# Autodesk Inventor assembly: Rotating Assembly
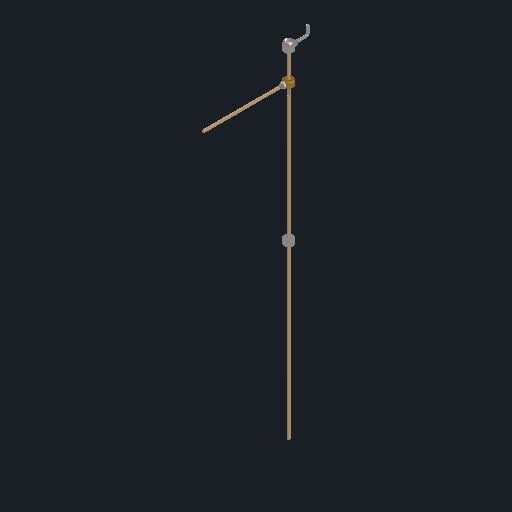
[picture p0: Inventor's stored thumbnail of the model, 512x512]
Saved by Autodesk Inventor 2027.1 (Build 311270010, 270A)
## iProperties
Created: 2025-09-16
Document SubType Name: Assembly
Designer: SD
Mass: 42.3595 g
Surface Area: 61.7875 cm^2
Volume: 4.97569 cm^3
Density: 8.51329 g/cm^3
Project: Automatic Tea Steeping mechanism
Part Number: Rotating Assembly
BOM-Mass: 0.04236
BOM-Area: 0.006
Author: SD
Title: Rotating Assembly
## Documents named in this file (9)
- C:\Users\Gamer\Documents\Projects\Auto Tea Steeper\Public Version\Automatic Tea Steeper\CAD\Workspace\Rotating Assembly.iam
- C:\Users\Gamer\Documents\Projects\Auto Tea Steeper\Public Version\Automatic Tea Steeper\CAD\Workspace\Rotating Rod 370mm.ipt
- C:\Users\Gamer\Documents\Projects\Auto Tea Steeper\Public Version\Automatic Tea Steeper\CAD\Workspace\Top Lock Cap.ipt
- C:\Users\Gamer\Documents\Projects\Auto Tea Steeper\Public Version\Automatic Tea Steeper\CAD\Workspace\Lock Handel.ipt
- C:\Users\Gamer\Documents\Projects\Auto Tea Steeper\Public Version\Automatic Tea Steeper\CAD\Workspace\Hardware\M3 Hex Nut.ipt
- C:\Users\Gamer\Documents\Projects\Auto Tea Steeper\Public Version\Automatic Tea Steeper\CAD\Workspace\Pendulum Arm Cap.ipt
- C:\Users\Gamer\Documents\Projects\Auto Tea Steeper\Public Version\Automatic Tea Steeper\CAD\Workspace\Pendulum Arm.ipt
- C:\Users\Gamer\Documents\Projects\Auto Tea Steeper\Public Version\Automatic Tea Steeper\CAD\Workspace\Lower Lock Cap.ipt
- C:\Users\Gamer\Documents\Projects\Auto Tea Steeper\Public Version\Automatic Tea Steeper\CAD\Workspace\Hardware\Grub Screw 3x3mm.ipt
## Components (9 placed, 8 different names)
1. Rotating Rod 370mm:1 — Flush:1, Mate:1, Mate:2, Mate:5, Mate:7, Mate:8, Mate:10, Mate:14, Mate:15, Mate:18
2. Top Lock Cap:1 — Mate:1, Mate:2, Mate:3, Mate:4
3. Lock Handel:1 — Mate:4, Mate:5, Flush:2, Mate:11, Mate:12
4. Pendulum Arm Cap:1 — Mate:7, Mate:8, Flush:3, Mate:9
5. Pendulum Arm:1 — Mate:9, Mate:10, Mate:13
6. M3 Hex Nut:1 — Mate:11, Mate:12
7. M3 Hex Nut:2 — Mate:13
8. Lower Lock Cap:1 — Mate:14, Mate:15, Mate:16, Mate:17
9. ISO 4026 M3 x 3:1 — Mate:17, Mate:18
## Relationships (20: Mate 17, Flush 3)
- Flush:1: Rotating Rod 370mm:1
- Mate:1: Rotating Rod 370mm:1 ↔ Top Lock Cap:1
- Mate:2 (-7 mm): Rotating Rod 370mm:1 ↔ Top Lock Cap:1
- Mate:3: Top Lock Cap:1
- Mate:4: Top Lock Cap:1 ↔ Lock Handel:1
- Mate:5: Rotating Rod 370mm:1 ↔ Lock Handel:1
- Flush:2: Lock Handel:1
- Mate:7: Rotating Rod 370mm:1 ↔ Pendulum Arm Cap:1
- Mate:8: Rotating Rod 370mm:1 ↔ Pendulum Arm Cap:1
- Flush:3: Pendulum Arm Cap:1
- Mate:9: Pendulum Arm Cap:1 ↔ Pendulum Arm:1
- Mate:10: Rotating Rod 370mm:1 ↔ Pendulum Arm:1
- Mate:11: Lock Handel:1 ↔ M3 Hex Nut:1
- Mate:12 (13.1 mm): Lock Handel:1 ↔ M3 Hex Nut:1
- Mate:13: Pendulum Arm:1 ↔ M3 Hex Nut:2
- Mate:14: Rotating Rod 370mm:1 ↔ Lower Lock Cap:1
- Mate:15: Rotating Rod 370mm:1 ↔ Lower Lock Cap:1
- Mate:16: Lower Lock Cap:1
- Mate:17: Lower Lock Cap:1 ↔ ISO 4026 M3 x 3:1
- Mate:18: Rotating Rod 370mm:1 ↔ ISO 4026 M3 x 3:1
